# Autodesk Inventor assembly: 100-00
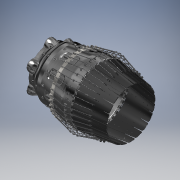
[picture p0: Inventor's stored thumbnail of the model, 180x180]
Saved by Autodesk Inventor 2019 (Build 230136000, 136)
## iProperties
Company: Autodesk Inc.
Created: 2017-03-17
Part Number: 100-00
Document SubType Name: Assembly
Designer: Autodesk Inc.
Mass: 10004.3 g
Surface Area: 12185.9 cm^2
Volume: 2054.88 cm^3
Density: 4.86856 g/cm^3
Author: Inventor
## Documents named in this file (11)
- C:\TEMP\Jet Engine Model\Workspace\Exhaust Assembly.iam
- C:\TEMP\Jet Engine Model\Workspace\Rear Casing.ipt
- C:\TEMP\Jet Engine Model\Workspace\Flare Base.ipt
- C:\TEMP\Jet Engine Model\Workspace\Flare Lever-3.ipt
- C:\TEMP\Jet Engine Model\Workspace\Flare Lever-1.ipt
- C:\TEMP\Jet Engine Model\Workspace\Flare Lever-2.ipt
- C:\TEMP\Jet Engine Model\Workspace\Heat Ring.ipt
- C:\TEMP\Jet Engine Model\Workspace\Blade-1.ipt
- C:\TEMP\Jet Engine Model\Workspace\Blade-2.ipt
- C:\TEMP\Jet Engine Model\Workspace\Blade-3.ipt
- C:\TEMP\Jet Engine Model\Libraries\Content Center Files\en-US\Rivet GB_T 1014-1986\Rivet GB_T 1014-1986-2 X 4.ipt
## Components (283 placed, 11 different names)
1. Rear Casing:1 — Mate:1, Insert:2, Mate:5, Mate:6, Flush:3, Flush:4, Mate:8, Flush:5, Mate:10, Insert:8, Mate:12
2. Flare Base:1 — Mate:1, Insert:1, Flush:5, Insert:7
3. Heat Ring:1 — Mate:5, Mate:8
4. Flare Lever-2:1 — Insert:1, Insert:3, Insert:5
5. Flare Lever-2:2 — Insert:7, Insert:9, Insert:10
6. Flare Lever-3:2 — Insert:8, Insert:9
7. Flare Lever-3:1 — Insert:2, Insert:3
8. Flare Lever-4:1 — Insert:5, Insert:6
9. Flare Lever-1:2 — Insert:10, Insert:11
10. Rivet GB/T 1014-1986 2 X 4:5 — Mate:17, Tangent:5
11. Rivet GB/T 1014-1986 2 X 4:4 — Mate:16, Tangent:4
12. Rivet GB/T 1014-1986 2 X 4:3 — Mate:15, Tangent:3
13. Rivet GB/T 1014-1986 2 X 4:2 — Mate:14, Tangent:2
14. Rivet GB/T 1014-1986 2 X 4:1 — Mate:13, Tangent:1
15. Blade-1:1 — Mate:9, Flush:6, Mate:11
16. Blade-2:1 — Mate:12, Insert:11
17. Blade-3:1 — Mate:9, Flush:6, Mate:10, Mate:11, Insert:6, Mate:13, Tangent:1, Mate:14, Tangent:2, Mate:15, Tangent:3, Mate:16, Mate:17, Tangent:4, Tangent:5
18. Flare Lever-2:3
19. Flare Lever-2:4
20. Flare Lever-3:3
21. Flare Lever-3:4
22. Flare Lever-1:3
23. Flare Lever-1:4
24. Rivet GB/T 1014-1986 2 X 4:184
25. Rivet GB/T 1014-1986 2 X 4:185
26. Rivet GB/T 1014-1986 2 X 4:186
27. Rivet GB/T 1014-1986 2 X 4:187
28. Rivet GB/T 1014-1986 2 X 4:188
29. Blade-1:2
30. Blade-2:2
31. Blade-3:2
32. Flare Lever-2:5
33. Flare Lever-2:6
34. Flare Lever-3:5
35. Flare Lever-3:6
36. Flare Lever-1:5
37. Flare Lever-1:6
38. Rivet GB/T 1014-1986 2 X 4:189
39. Rivet GB/T 1014-1986 2 X 4:190
40. Rivet GB/T 1014-1986 2 X 4:191
41. Rivet GB/T 1014-1986 2 X 4:192
42. Rivet GB/T 1014-1986 2 X 4:193
43. Blade-1:3
44. Blade-2:3
45. Blade-3:3
46. Flare Lever-2:7
47. Flare Lever-2:8
48. Flare Lever-3:7
49. Flare Lever-3:8
50. Flare Lever-1:7
51. Flare Lever-1:8
52. Rivet GB/T 1014-1986 2 X 4:194
53. Rivet GB/T 1014-1986 2 X 4:195
54. Rivet GB/T 1014-1986 2 X 4:196
55. Rivet GB/T 1014-1986 2 X 4:197
56. Rivet GB/T 1014-1986 2 X 4:198
57. Blade-1:4
58. Blade-2:4
59. Blade-3:4
60. Flare Lever-2:9
61. Flare Lever-2:10
62. Flare Lever-3:9
63. Flare Lever-3:10
64. Flare Lever-1:9
65. Flare Lever-1:10
66. Rivet GB/T 1014-1986 2 X 4:199
67. Rivet GB/T 1014-1986 2 X 4:200
68. Rivet GB/T 1014-1986 2 X 4:201
69. Rivet GB/T 1014-1986 2 X 4:202
70. Rivet GB/T 1014-1986 2 X 4:203
71. Blade-1:5
72. Blade-2:5
73. Blade-3:5
74. Flare Lever-2:11
75. Flare Lever-2:12
76. Flare Lever-3:11
77. Flare Lever-3:12
78. Flare Lever-1:11
79. Flare Lever-1:12
80. Rivet GB/T 1014-1986 2 X 4:204
81. Rivet GB/T 1014-1986 2 X 4:205
82. Rivet GB/T 1014-1986 2 X 4:206
83. Rivet GB/T 1014-1986 2 X 4:207
84. Rivet GB/T 1014-1986 2 X 4:208
85. Blade-1:6
86. Blade-2:6
87. Blade-3:6
88. Flare Lever-2:13
89. Flare Lever-2:14
90. Flare Lever-3:13
91. Flare Lever-3:14
92. Flare Lever-1:13
93. Flare Lever-1:14
94. Rivet GB/T 1014-1986 2 X 4:209
95. Rivet GB/T 1014-1986 2 X 4:210
96. Rivet GB/T 1014-1986 2 X 4:211
97. Rivet GB/T 1014-1986 2 X 4:212
98. Rivet GB/T 1014-1986 2 X 4:213
99. Blade-1:7
100. Blade-2:7
101. Blade-3:7
102. Flare Lever-2:15
103. Flare Lever-2:16
104. Flare Lever-3:15
105. Flare Lever-3:16
106. Flare Lever-1:15
107. Flare Lever-1:16
108. Rivet GB/T 1014-1986 2 X 4:214
109. Rivet GB/T 1014-1986 2 X 4:215
110. Rivet GB/T 1014-1986 2 X 4:216
111. Rivet GB/T 1014-1986 2 X 4:217
112. Rivet GB/T 1014-1986 2 X 4:218
113. Blade-1:8
114. Blade-2:8
115. Blade-3:8
116. Flare Lever-2:17
117. Flare Lever-2:18
118. Flare Lever-3:17
119. Flare Lever-3:18
120. Flare Lever-1:17
121. Flare Lever-1:18
122. Rivet GB/T 1014-1986 2 X 4:219
123. Rivet GB/T 1014-1986 2 X 4:220
124. Rivet GB/T 1014-1986 2 X 4:221
125. Rivet GB/T 1014-1986 2 X 4:222
126. Rivet GB/T 1014-1986 2 X 4:223
127. Blade-1:9
128. Blade-2:9
129. Blade-3:9
130. Flare Lever-2:19
131. Flare Lever-2:20
132. Flare Lever-3:19
133. Flare Lever-3:20
134. Flare Lever-1:19
135. Flare Lever-1:20
136. Rivet GB/T 1014-1986 2 X 4:224
137. Rivet GB/T 1014-1986 2 X 4:225
138. Rivet GB/T 1014-1986 2 X 4:226
139. Rivet GB/T 1014-1986 2 X 4:227
140. Rivet GB/T 1014-1986 2 X 4:228
141. Blade-1:10
142. Blade-2:10
143. Blade-3:10
144. Flare Lever-2:21
145. Flare Lever-2:22
146. Flare Lever-3:21
147. Flare Lever-3:22
148. Flare Lever-1:21
149. Flare Lever-1:22
150. Rivet GB/T 1014-1986 2 X 4:229
151. Rivet GB/T 1014-1986 2 X 4:230
152. Rivet GB/T 1014-1986 2 X 4:231
153. Rivet GB/T 1014-1986 2 X 4:232
154. Rivet GB/T 1014-1986 2 X 4:233
155. Blade-1:11
156. Blade-2:11
157. Blade-3:11
158. Flare Lever-2:23
159. Flare Lever-2:24
160. Flare Lever-3:23
161. Flare Lever-3:24
162. Flare Lever-1:23
163. Flare Lever-1:24
164. Rivet GB/T 1014-1986 2 X 4:234
165. Rivet GB/T 1014-1986 2 X 4:235
166. Rivet GB/T 1014-1986 2 X 4:236
167. Rivet GB/T 1014-1986 2 X 4:237
168. Rivet GB/T 1014-1986 2 X 4:238
169. Blade-1:12
170. Blade-2:12
171. Blade-3:12
172. Flare Lever-2:25
173. Flare Lever-2:26
174. Flare Lever-3:25
175. Flare Lever-3:26
176. Flare Lever-1:25
177. Flare Lever-1:26
178. Rivet GB/T 1014-1986 2 X 4:239
179. Rivet GB/T 1014-1986 2 X 4:240
180. Rivet GB/T 1014-1986 2 X 4:241
181. Rivet GB/T 1014-1986 2 X 4:242
182. Rivet GB/T 1014-1986 2 X 4:243
183. Blade-1:13
184. Blade-2:13
185. Blade-3:13
186. Flare Lever-2:27
187. Flare Lever-2:28
188. Flare Lever-3:27
189. Flare Lever-3:28
190. Flare Lever-1:27
191. Flare Lever-1:28
192. Rivet GB/T 1014-1986 2 X 4:244
193. Rivet GB/T 1014-1986 2 X 4:245
194. Rivet GB/T 1014-1986 2 X 4:246
195. Rivet GB/T 1014-1986 2 X 4:247
196. Rivet GB/T 1014-1986 2 X 4:248
197. Blade-1:14
198. Blade-2:14
199. Blade-3:14
200. Flare Lever-2:29
201. Flare Lever-2:30
202. Flare Lever-3:29
203. Flare Lever-3:30
204. Flare Lever-1:29
205. Flare Lever-1:30
206. Rivet GB/T 1014-1986 2 X 4:249
207. Rivet GB/T 1014-1986 2 X 4:250
208. Rivet GB/T 1014-1986 2 X 4:251
209. Rivet GB/T 1014-1986 2 X 4:252
210. Rivet GB/T 1014-1986 2 X 4:253
211. Blade-1:15
212. Blade-2:15
213. Blade-3:15
214. Flare Lever-2:31
215. Flare Lever-2:32
216. Flare Lever-3:31
217. Flare Lever-3:32
218. Flare Lever-1:31
219. Flare Lever-1:32
220. Rivet GB/T 1014-1986 2 X 4:254
221. Rivet GB/T 1014-1986 2 X 4:255
222. Rivet GB/T 1014-1986 2 X 4:256
223. Rivet GB/T 1014-1986 2 X 4:257
224. Rivet GB/T 1014-1986 2 X 4:258
225. Blade-1:16
226. Blade-2:16
227. Blade-3:16
228. Flare Lever-2:33
229. Flare Lever-2:34
230. Flare Lever-3:33
231. Flare Lever-3:34
232. Flare Lever-1:33
233. Flare Lever-1:34
234. Rivet GB/T 1014-1986 2 X 4:259
235. Rivet GB/T 1014-1986 2 X 4:260
236. Rivet GB/T 1014-1986 2 X 4:261
237. Rivet GB/T 1014-1986 2 X 4:262
238. Rivet GB/T 1014-1986 2 X 4:263
239. Blade-1:17
240. Blade-2:17
241. Blade-3:17
242. Flare Lever-2:35
243. Flare Lever-2:36
244. Flare Lever-3:35
245. Flare Lever-3:36
246. Flare Lever-1:35
247. Flare Lever-1:36
248. Rivet GB/T 1014-1986 2 X 4:264
249. Rivet GB/T 1014-1986 2 X 4:265
250. Rivet GB/T 1014-1986 2 X 4:266
251. Rivet GB/T 1014-1986 2 X 4:267
252. Rivet GB/T 1014-1986 2 X 4:268
253. Blade-1:18
254. Blade-2:18
255. Blade-3:18
256. Flare Lever-2:37
257. Flare Lever-2:38
258. Flare Lever-3:37
259. Flare Lever-3:38
260. Flare Lever-1:37
261. Flare Lever-1:38
262. Rivet GB/T 1014-1986 2 X 4:269
263. Rivet GB/T 1014-1986 2 X 4:270
264. Rivet GB/T 1014-1986 2 X 4:271
265. Rivet GB/T 1014-1986 2 X 4:272
266. Rivet GB/T 1014-1986 2 X 4:273
267. Blade-1:19
268. Blade-2:19
269. Blade-3:19
270. Flare Lever-2:39
271. Flare Lever-2:40
272. Flare Lever-3:39
273. Flare Lever-3:40
274. Flare Lever-1:39
275. Flare Lever-1:40
276. Rivet GB/T 1014-1986 2 X 4:274
277. Rivet GB/T 1014-1986 2 X 4:275
278. Rivet GB/T 1014-1986 2 X 4:276
279. Rivet GB/T 1014-1986 2 X 4:277
280. Rivet GB/T 1014-1986 2 X 4:278
281. Blade-1:20
282. Blade-2:20
283. Blade-3:20
## Component patterns: (20 elements, first: Flare Lever-2:1 + Flare Lever-2:2 + Flare Lever-3:2 + Flare Lever-3:1 + Flare Lever-4:1 + Flare Lever-1:2 + Rivet GB/T 1014-1986 2 X 4:5 + Rivet GB/T 1014-1986 2 X 4:4 + Rivet GB/T 1014-1986 2 X 4:3 + Rivet GB/T 1014-1986 2 X 4:2 + Rivet GB/T 1014-1986 2 X 4:1 + Blade-1:1 + Blade-2:1 + Blade-3:1)
## Relationships (32: Mate 13, Insert 10, Tangent 5, Flush 4)
- Mate:1: Rear Casing:1 ↔ Flare Base:1
- Insert:1: Flare Base:1 ↔ Flare Lever-2:1
- Insert:2: Rear Casing:1 ↔ Flare Lever-3:1
- Insert:3: Flare Lever-2:1 ↔ Flare Lever-3:1
- Insert:5: Flare Lever-2:1 ↔ Flare Lever-4:1
- Mate:5: Rear Casing:1 ↔ Heat Ring:1
- Mate:6: Rear Casing:1
- Flush:3: Rear Casing:1
- Flush:4: Rear Casing:1
- Mate:8 (80 mm): Rear Casing:1 ↔ Heat Ring:1
- Flush:5 (11 mm): Rear Casing:1 ↔ Flare Base:1
- Mate:9: Blade-1:1 ↔ Blade-3:1
- Flush:6: Blade-1:1 ↔ Blade-3:1
- Mate:10: Rear Casing:1 ↔ Blade-3:1
- Mate:11: Blade-1:1 ↔ Blade-3:1
- Insert:6: Flare Lever-4:1 ↔ Blade-3:1
- Insert:7: Flare Base:1 ↔ Flare Lever-2:2
- Insert:8: Rear Casing:1 ↔ Flare Lever-3:2
- Insert:9: Flare Lever-2:2 ↔ Flare Lever-3:2
- Insert:10: Flare Lever-2:2 ↔ Flare Lever-1:2
- Mate:12: Rear Casing:1 ↔ Blade-2:1
- Insert:11: Flare Lever-1:2 ↔ Blade-2:1
- Mate:13: Rivet GB/T 1014-1986 2 X 4:1 ↔ Blade-3:1
- Tangent:1 (0.1 mm): Rivet GB/T 1014-1986 2 X 4:1 ↔ Blade-3:1
- Mate:14: Rivet GB/T 1014-1986 2 X 4:2 ↔ Blade-3:1
- Tangent:2 (0.1 mm): Rivet GB/T 1014-1986 2 X 4:2 ↔ Blade-3:1
- Mate:15: Rivet GB/T 1014-1986 2 X 4:3 ↔ Blade-3:1
- Tangent:3 (0.1 mm): Rivet GB/T 1014-1986 2 X 4:3 ↔ Blade-3:1
- Mate:16: Rivet GB/T 1014-1986 2 X 4:4 ↔ Blade-3:1
- Mate:17: Rivet GB/T 1014-1986 2 X 4:5 ↔ Blade-3:1
- Tangent:4 (0.1 mm): Rivet GB/T 1014-1986 2 X 4:4 ↔ Blade-3:1
- Tangent:5 (0.1 mm): Rivet GB/T 1014-1986 2 X 4:5 ↔ Blade-3:1
